# Autodesk Inventor assembly: estufa morango 20
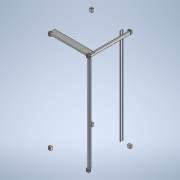
[picture p0: Inventor's stored thumbnail of the model, 180x180]
Saved by Autodesk Inventor 2020 (Build 240168000, 168)
## iProperties
Created: 2022-10-16
Part Number: estufa morango 20
Document SubType Name: Assembly
Designer: super
Author: super
## Documents named in this file (6)
- C:\desk\promissionsave\inventor\container\estufa morango 20.iam
- C:\desk\promissionsave\inventor\container\c150x43x15.ipt
- C:\desk\promissionsave\inventor\container\corners 20feet.iam
- C:\desk\promissionsave\inventor\container\c lateral struct.ipt
- C:\desk\promissionsave\inventor\container\pilar.ipt
- C:\desk\promissionsave\inventor\container\Part2.ipt
## Components (5 placed, 5 different names)
1. c150x43x15:1
2. corners 20feet:1 [sub-assembly] — Mate:1, Mate:2, Flush:1, Mate:3, Flush:2, Flush:3
3. c lateral struct:1
4. pilar:1 — Mate:3, Flush:2, Flush:5, Mate:7
5. Part2:1 — Flush:3, Flush:5, Mate:7
## Relationships (8: Mate 4, Flush 4)
- Mate:1: corners 20feet:1
- Mate:2: corners 20feet:1
- Flush:1: corners 20feet:1
- Mate:3: corners 20feet:1 ↔ pilar:1
- Flush:2: corners 20feet:1 ↔ pilar:1
- Flush:3: corners 20feet:1 ↔ Part2:1
- Flush:5: pilar:1 ↔ Part2:1
- Mate:7: pilar:1 ↔ Part2:1
